# Autodesk Inventor assembly: am-2557 Nano Tube 20 three 500 key shafts - 2 motor inputs
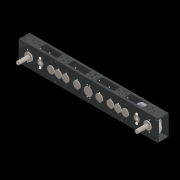
[picture p0: Inventor's stored thumbnail of the model, 180x180]
Saved by Autodesk Inventor 2022 (Build 260153000, 153)
## iProperties
Created: 2017-01-24
Part Number: am-2557 Nano Tube 20 three 500 key shafts - 2 motor inputs
Description: STEP AP214
Document SubType Name: Assembly
Designer: timmy
Sending System: SolidWorks 2014
Preprocessor: SwSTEP 2.0
Title: am-2257 Nano Tube 20 three 500 key shafts - 2 motor inputs.STEP
Revision Number: ANY
## Documents named in this file (16)
- S:\Inventor\RoboCatz\T-Shirt\am-2557 Nano Tube 20 three 500 key shafts - 2 motor inputs.iam
- S:\Inventor\RoboCatz\T-Shirt\NanoTube20 3-outputV3.ipt
- S:\Inventor\RoboCatz\T-Shirt\FR8ZZ Hex Bearing.ipt
- S:\Inventor\RoboCatz\T-Shirt\FR6ZZ-L Bearing.ipt
- S:\Inventor\RoboCatz\T-Shirt\Toughbox Nano d04 am-0506.ipt
- S:\Inventor\RoboCatz\T-Shirt\Spacer am-1151.ipt
- S:\Inventor\RoboCatz\T-Shirt\500-e-klip.ipt
- S:\Inventor\RoboCatz\T-Shirt\FR6.ipt
- S:\Inventor\RoboCatz\T-Shirt\R6ZZ Bearing.ipt
- S:\Inventor\RoboCatz\T-Shirt\Toughbox d07.ipt
- S:\Inventor\RoboCatz\T-Shirt\Toughbox 14T Small Cluster.ipt
- S:\Inventor\RoboCatz\T-Shirt\Toughbox 50T Large Cluster.ipt
- S:\Inventor\RoboCatz\T-Shirt\Toughbox 50T Output.ipt
- S:\Inventor\RoboCatz\T-Shirt\BHCS 10-32 x 0.375_SBHCSCREW 0.19-32x0.5-HX-C.ipt
- S:\Inventor\RoboCatz\T-Shirt\am-2986 FR8ZZ Hex Bearing.ipt
- S:\Inventor\RoboCatz\T-Shirt\plug1.ipt
## Components (35 placed, 28 different names)
1. NanoTube20 3-outputV3_1 — Mate:1, Mate:2, Mate:3, Mate:4, Mate:5, Mate:6, Mate:7, Mate:8, Mate:9, Mate:10, Mate:11, Mate:12, Mate:13, Mate:14, Mate:15, Mate:16, Mate:17, Mate:18
2. FR8ZZ Hex Bearing_2
3. FR6ZZ-L Bearing_3
4. Toughbox Nano d04 am-0506_4
5. Spacer am-1151_5
6. 500-e-klip_6
7. FR6_7
8. R6ZZ Bearing_8
9. Toughbox d07_9
10. Toughbox 14T Small Cluster_10
11. Toughbox 50T Output_12
12. BHCS 10-32 x 0.375_SBHCSCREW 0.19-32x0.5-HX-C_13
13. BHCS 10-32 x 0.375_SBHCSCREW 0.19-32x0.5-HX-C_14
14. FR8ZZ Hex Bearing_40
15. FR6ZZ-L Bearing_41
16. Toughbox Nano d04 am-0506_42
17. Spacer am-1151_43
18. 500-e-klip_44
19. FR6_45
20. R6ZZ Bearing_46
21. Toughbox d07_47
22. Toughbox 14T Small Cluster_48
23. Toughbox 50T Large Cluster_49
24. Toughbox 50T Output_50
25. BHCS 10-32 x 0.375_SBHCSCREW 0.19-32x0.5-HX-C_51
26. BHCS 10-32 x 0.375_SBHCSCREW 0.19-32x0.5-HX-C_52
27. am-2986 FR8ZZ Hex Bearing:1 — Mate:1
28. plug1:1 — Mate:2, Mate:5, Mate:8
29. plug1:2 — Mate:3, Mate:4
30. plug1:3 — Mate:6, Mate:7
31. plug1:4 — Mate:9, Mate:12
32. plug1:5 — Mate:10, Mate:13
33. plug1:6 — Mate:11, Mate:14
34. plug1:10 — Mate:15, Mate:16
35. plug1:11 — Mate:17, Mate:18
## Relationships (18: Mate 18)
- Mate:1: NanoTube20 3-outputV3_1 ↔ am-2986 FR8ZZ Hex Bearing:1
- Mate:2: NanoTube20 3-outputV3_1 ↔ plug1:1
- Mate:3: NanoTube20 3-outputV3_1 ↔ plug1:2
- Mate:4: NanoTube20 3-outputV3_1 ↔ plug1:2
- Mate:5: NanoTube20 3-outputV3_1 ↔ plug1:1
- Mate:6: NanoTube20 3-outputV3_1 ↔ plug1:3
- Mate:7: NanoTube20 3-outputV3_1 ↔ plug1:3
- Mate:8: NanoTube20 3-outputV3_1 ↔ plug1:1
- Mate:9: NanoTube20 3-outputV3_1 ↔ plug1:4
- Mate:10: NanoTube20 3-outputV3_1 ↔ plug1:5
- Mate:11: NanoTube20 3-outputV3_1 ↔ plug1:6
- Mate:12: NanoTube20 3-outputV3_1 ↔ plug1:4
- Mate:13: NanoTube20 3-outputV3_1 ↔ plug1:5
- Mate:14: NanoTube20 3-outputV3_1 ↔ plug1:6
- Mate:15: NanoTube20 3-outputV3_1 ↔ plug1:10
- Mate:16: NanoTube20 3-outputV3_1 ↔ plug1:10
- Mate:17: NanoTube20 3-outputV3_1 ↔ plug1:11
- Mate:18: NanoTube20 3-outputV3_1 ↔ plug1:11
